# Autodesk Inventor assembly: КВ33.044.200 - Каретка оси Х
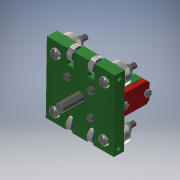
[picture p0: Inventor's stored thumbnail of the model, 180x180]
Saved by Autodesk Inventor 2019 (Build 230136000, 136)
## iProperties
Created: 2019-07-16
Part Number: КВ33.044.200 - Каретка оси Х
Material: Типовые
Document SubType Name: Assembly
Designer: Петров Иван
Author: Петров Иван
## Documents named in this file (14)
- E:\IVAN\Kvantoriada2019\optimal_gripper\hardware\КВ33.044.200 - Каретка оси Х.iam
- E:\IVAN\Kvantoriada2019\optimal_gripper\hardware\КВ33.044.201 - Щека каретки.ipt
- E:\IVAN\Kvantoriada2019\optimal_gripper\hardware\Стандартные изделия\Подшипник 626Z.ipt
- E:\IVAN\Kvantoriada2019\optimal_gripper\hardware\Стандартные изделия\Подшипник 624Z.ipt
- E:\IVAN\Kvantoriada2019\optimal_gripper\hardware\КВ33.044.203 - Прижим ремня.ipt
- E:\IVAN\Kvantoriada2019\optimal_gripper\hardware\Стандартные изделия\Винт М8х25 с потайной головкой.ipt
- E:\IVAN\Kvantoriada2019\optimal_gripper\hardware\Стандартные изделия\Винт М5х10 с потайной головкой.ipt
- C:\Users\Петров Иван\Documents\Inventor\Content Center Files\R2019\ru-RU\AS 1427(10)\AS 1427 - M4 x 35(7).ipt
- C:\Users\Петров Иван\Documents\Inventor\Content Center Files\R2019\ru-RU\JIS B 1101(1)\JIS B 1101 - M5 x 30(2).ipt
- C:\Users\Петров Иван\Documents\Inventor\Content Center Files\R2019\ru-RU\AS 1237 (2.1)\AS 1237 - 6.ipt
- C:\Users\Петров Иван\Documents\Inventor\Content Center Files\R2019\ru-RU\AS 1237 (2.1)\AS 1237 - 5.ipt
- C:\Users\Петров Иван\Documents\Inventor\Content Center Files\R2019\ru-RU\ANSI B18.2.4.2M\ANSI B18.2.4.2M - M5x0,8 - 8.ipt
- C:\Users\Петров Иван\Documents\Inventor\Content Center Files\R2019\ru-RU\JIS B 1101(4)\JIS B 1101 - M3 x 12(3).ipt
- C:\Users\Петров Иван\Documents\Inventor\Content Center Files\R2019\ru-RU\BS EN 24032\ISO 4032 - M3BS EN.ipt
## Components (37 placed, 13 different names)
1. КВ33.044.201 - Щека каретки:1 — Совмещение:1, Совмещение:2, Совмещение:3, Совмещение:4, Совмещение:5, Совмещение:6, Совмещение:7, Совмещение:8, Совмещение:9, Совмещение:10, Совмещение:11, Совмещение:12, Совмещение:13, Совмещение:14, Совмещение:15, Совмещение:16, Совмещение:17, Совмещение:18, Совмещение:19, Совмещение:20, Заподлицо:1, Совмещение:21, Совмещение:22, Совмещение:23, Совмещение:24, Заподлицо:2, Заподлицо:3, Заподлицо:4, Заподлицо:5, Совмещение:25, Совмещение:26, Совмещение:27, Совмещение:28, Вставка:1, Вставка:2, Вставка:3, Вставка:4, Вставка:5, Вставка:6, Вставка:7, Вставка:8, Совмещение:37, Совмещение:38, Совмещение:39, Совмещение:40
2. Подшипник 626Z:1 — Совмещение:1, Совмещение:8, Совмещение:34
3. Подшипник 626Z:2 — Совмещение:2, Совмещение:5, Совмещение:32
4. Подшипник 626Z:3 — Совмещение:3, Совмещение:7, Совмещение:36
5. Подшипник 626Z:4 — Совмещение:4, Совмещение:6, Совмещение:30
6. Подшипник 624Z:1 — Совмещение:9, Совмещение:10
7. Подшипник 624Z:2 — Совмещение:13, Совмещение:14
8. Подшипник 624Z:3 — Совмещение:11, Совмещение:12
9. Подшипник 624Z:4 — Совмещение:15, Совмещение:16
10. КВ33.044.203 - Прижим ремня:1 — Совмещение:17, Совмещение:18, Совмещение:19, Вставка:13, Вставка:14
11. Винт М8х25 с потайной головкой:1 — Совмещение:20, Заподлицо:1
12. Винт М5х10 с потайной головкой:1 — Совмещение:22, Заподлицо:2
13. Винт М5х10 с потайной головкой:2 — Совмещение:24, Заподлицо:3
14. Винт М5х10 с потайной головкой:3 — Совмещение:21, Заподлицо:5
15. Винт М5х10 с потайной головкой:4 — Совмещение:23, Заподлицо:4
16. AS 1427 (8) - метрическая M4 x 35:1 — Совмещение:25, Совмещение:26
17. AS 1427 (8) - метрическая M4 x 35:2 — Совмещение:27, Совмещение:28
18. JIS B 1101 - метрическая M5 x 30:1 — Вставка:1, Совмещение:33
19. JIS B 1101 - метрическая M5 x 30:2 — Вставка:2, Совмещение:35
20. JIS B 1101 - метрическая M5 x 30:3 — Вставка:3, Совмещение:29
21. JIS B 1101 - метрическая M5 x 30:4 — Вставка:4, Совмещение:31
22. AS 1237 (2.1) 6:1 — Вставка:5
23. AS 1237 (2.1) 6:2 — Вставка:6
24. AS 1237 (2.1) 6:3 — Вставка:7
25. AS 1237 (2.1) 6:4 — Вставка:8
26. AS 1237 (2.1) 5:1 — Совмещение:29, Совмещение:30, Вставка:10
27. AS 1237 (2.1) 5:2 — Совмещение:31, Совмещение:32, Вставка:9
28. AS 1237 (2.1) 5:3 — Совмещение:33, Совмещение:34, Вставка:11
29. AS 1237 (2.1) 5:4 — Совмещение:35, Совмещение:36, Вставка:12
30. ANSI B18.2.4.2M M5x0,8:1 — Вставка:9
31. ANSI B18.2.4.2M M5x0,8:2 — Вставка:10
32. ANSI B18.2.4.2M M5x0,8:3 — Вставка:11
33. ANSI B18.2.4.2M M5x0,8:4 — Вставка:12
34. JIS B 1101 - согласно ISO 1580 - метрическая M3 x 12:1 — Совмещение:37, Совмещение:38
35. JIS B 1101 - согласно ISO 1580 - метрическая M3 x 12:2 — Совмещение:39, Совмещение:40
36. BS EN 24032 - метрическая M3:1 — Вставка:13
37. BS EN 24032 - метрическая M3:2 — Вставка:14
## Relationships (59: Mate 40, Insert 14, Flush 5)
- Совмещение:1 [Mate]: КВ33.044.201 - Щека каретки:1 ↔ Подшипник 626Z:1
- Совмещение:2 [Mate]: КВ33.044.201 - Щека каретки:1 ↔ Подшипник 626Z:2
- Совмещение:3 [Mate]: КВ33.044.201 - Щека каретки:1 ↔ Подшипник 626Z:3
- Совмещение:4 [Mate]: КВ33.044.201 - Щека каретки:1 ↔ Подшипник 626Z:4
- Совмещение:5 [Mate] (1 mm): КВ33.044.201 - Щека каретки:1 ↔ Подшипник 626Z:2
- Совмещение:6 [Mate] (1 mm): КВ33.044.201 - Щека каретки:1 ↔ Подшипник 626Z:4
- Совмещение:7 [Mate] (1 mm): КВ33.044.201 - Щека каретки:1 ↔ Подшипник 626Z:3
- Совмещение:8 [Mate] (1 mm): КВ33.044.201 - Щека каретки:1 ↔ Подшипник 626Z:1
- Совмещение:9 [Mate]: КВ33.044.201 - Щека каретки:1 ↔ Подшипник 624Z:1
- Совмещение:10 [Mate] (0.5 mm): КВ33.044.201 - Щека каретки:1 ↔ Подшипник 624Z:1
- Совмещение:11 [Mate]: КВ33.044.201 - Щека каретки:1 ↔ Подшипник 624Z:3
- Совмещение:12 [Mate] (0.5 mm): КВ33.044.201 - Щека каретки:1 ↔ Подшипник 624Z:3
- Совмещение:13 [Mate]: КВ33.044.201 - Щека каретки:1 ↔ Подшипник 624Z:2
- Совмещение:14 [Mate] (0.5 mm): КВ33.044.201 - Щека каретки:1 ↔ Подшипник 624Z:2
- Совмещение:15 [Mate]: КВ33.044.201 - Щека каретки:1 ↔ Подшипник 624Z:4
- Совмещение:16 [Mate] (0.5 mm): КВ33.044.201 - Щека каретки:1 ↔ Подшипник 624Z:4
- Совмещение:17 [Mate]: КВ33.044.201 - Щека каретки:1 ↔ КВ33.044.203 - Прижим ремня:1
- Совмещение:18 [Mate]: КВ33.044.201 - Щека каретки:1 ↔ КВ33.044.203 - Прижим ремня:1
- Совмещение:19 [Mate]: КВ33.044.201 - Щека каретки:1 ↔ КВ33.044.203 - Прижим ремня:1
- Совмещение:20 [Mate]: КВ33.044.201 - Щека каретки:1 ↔ Винт М8х25 с потайной головкой:1
- Заподлицо:1 [Flush] (2 mm): КВ33.044.201 - Щека каретки:1 ↔ Винт М8х25 с потайной головкой:1
- Совмещение:21 [Mate]: КВ33.044.201 - Щека каретки:1 ↔ Винт М5х10 с потайной головкой:3
- Совмещение:22 [Mate]: КВ33.044.201 - Щека каретки:1 ↔ Винт М5х10 с потайной головкой:1
- Совмещение:23 [Mate]: КВ33.044.201 - Щека каретки:1 ↔ Винт М5х10 с потайной головкой:4
- Совмещение:24 [Mate]: КВ33.044.201 - Щека каретки:1 ↔ Винт М5х10 с потайной головкой:2
- Заподлицо:2 [Flush] (1 mm): КВ33.044.201 - Щека каретки:1 ↔ Винт М5х10 с потайной головкой:1
- Заподлицо:3 [Flush] (1 mm): КВ33.044.201 - Щека каретки:1 ↔ Винт М5х10 с потайной головкой:2
- Заподлицо:4 [Flush] (1 mm): КВ33.044.201 - Щека каретки:1 ↔ Винт М5х10 с потайной головкой:4
- Заподлицо:5 [Flush] (1 mm): КВ33.044.201 - Щека каретки:1 ↔ Винт М5х10 с потайной головкой:3
- Совмещение:25 [Mate]: КВ33.044.201 - Щека каретки:1 ↔ AS 1427 (8) - метрическая M4 x 35:1
- Совмещение:26 [Mate]: КВ33.044.201 - Щека каретки:1 ↔ AS 1427 (8) - метрическая M4 x 35:1
- Совмещение:27 [Mate]: КВ33.044.201 - Щека каретки:1 ↔ AS 1427 (8) - метрическая M4 x 35:2
- Совмещение:28 [Mate]: КВ33.044.201 - Щека каретки:1 ↔ AS 1427 (8) - метрическая M4 x 35:2
- Вставка:1 [Insert]: КВ33.044.201 - Щека каретки:1 ↔ JIS B 1101 - метрическая M5 x 30:1
- Вставка:2 [Insert]: КВ33.044.201 - Щека каретки:1 ↔ JIS B 1101 - метрическая M5 x 30:2
- Вставка:3 [Insert]: КВ33.044.201 - Щека каретки:1 ↔ JIS B 1101 - метрическая M5 x 30:3
- Вставка:4 [Insert]: КВ33.044.201 - Щека каретки:1 ↔ JIS B 1101 - метрическая M5 x 30:4
- Вставка:5 [Insert]: КВ33.044.201 - Щека каретки:1 ↔ AS 1237 (2.1) 6:1
- Вставка:6 [Insert]: КВ33.044.201 - Щека каретки:1 ↔ AS 1237 (2.1) 6:2
- Вставка:7 [Insert]: КВ33.044.201 - Щека каретки:1 ↔ AS 1237 (2.1) 6:3
- Вставка:8 [Insert]: КВ33.044.201 - Щека каретки:1 ↔ AS 1237 (2.1) 6:4
- Совмещение:29 [Mate]: JIS B 1101 - метрическая M5 x 30:3 ↔ AS 1237 (2.1) 5:1
- Совмещение:30 [Mate]: Подшипник 626Z:4 ↔ AS 1237 (2.1) 5:1
- Совмещение:31 [Mate]: JIS B 1101 - метрическая M5 x 30:4 ↔ AS 1237 (2.1) 5:2
- Совмещение:32 [Mate]: Подшипник 626Z:2 ↔ AS 1237 (2.1) 5:2
- Совмещение:33 [Mate]: JIS B 1101 - метрическая M5 x 30:1 ↔ AS 1237 (2.1) 5:3
- Совмещение:34 [Mate]: Подшипник 626Z:1 ↔ AS 1237 (2.1) 5:3
- Совмещение:35 [Mate]: JIS B 1101 - метрическая M5 x 30:2 ↔ AS 1237 (2.1) 5:4
- Совмещение:36 [Mate]: Подшипник 626Z:3 ↔ AS 1237 (2.1) 5:4
- Вставка:9 [Insert]: AS 1237 (2.1) 5:2 ↔ ANSI B18.2.4.2M M5x0,8:1
- Вставка:10 [Insert]: AS 1237 (2.1) 5:1 ↔ ANSI B18.2.4.2M M5x0,8:2
- Вставка:11 [Insert]: AS 1237 (2.1) 5:3 ↔ ANSI B18.2.4.2M M5x0,8:3
- Вставка:12 [Insert]: AS 1237 (2.1) 5:4 ↔ ANSI B18.2.4.2M M5x0,8:4
- Совмещение:37 [Mate]: КВ33.044.201 - Щека каретки:1 ↔ JIS B 1101 - согласно ISO 1580 - метрическая M3 x 12:1
- Совмещение:38 [Mate]: КВ33.044.201 - Щека каретки:1 ↔ JIS B 1101 - согласно ISO 1580 - метрическая M3 x 12:1
- Совмещение:39 [Mate]: КВ33.044.201 - Щека каретки:1 ↔ JIS B 1101 - согласно ISO 1580 - метрическая M3 x 12:2
- Совмещение:40 [Mate]: КВ33.044.201 - Щека каретки:1 ↔ JIS B 1101 - согласно ISO 1580 - метрическая M3 x 12:2
- Вставка:13 [Insert]: КВ33.044.203 - Прижим ремня:1 ↔ BS EN 24032 - метрическая M3:1
- Вставка:14 [Insert]: КВ33.044.203 - Прижим ремня:1 ↔ BS EN 24032 - метрическая M3:2
